# Autodesk Inventor assembly: Cart Assembly
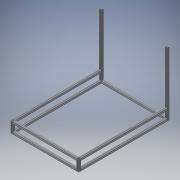
[picture p0: Inventor's stored thumbnail of the model, 180x180]
Saved by Autodesk Inventor 2016 SP2 (Build 200236200, 236)
## iProperties
Created: 2018-02-07
Part Number: Cart Assembly
Document SubType Name: Assembly
Designer: CAD
Author: CAD
## Documents named in this file (5)
- C:\Users\CAD\Documents\GitHub\FIRST-ROBOTICS-2018-5436-CAD\Cart\Cart Assembly.iam
- C:\Users\CAD\Documents\GitHub\FIRST-ROBOTICS-2018-5436-CAD\Cart\Horizontal width piece.ipt
- C:\Users\CAD\Documents\GitHub\FIRST-ROBOTICS-2018-5436-CAD\Cart\Horizontal pice.ipt
- C:\Users\CAD\Documents\GitHub\FIRST-ROBOTICS-2018-5436-CAD\Cart\Vertical piece Handle side.ipt
- C:\Users\CAD\Documents\GitHub\FIRST-ROBOTICS-2018-5436-CAD\Cart\Vertical Piece front side.ipt
## Components (11 placed, 4 different names)
1. Horizontal width piece:1 — Flush:13, Flush:14, Flush:15, Mate:8
2. Horizontal width piece:2 — Mate:2, Flush:3, Flush:4, Flush:5, Flush:6, Mate:3, Flush:8
3. Horizontal pice:1 — Mate:1, Flush:1, Flush:2, Flush:4, Mate:6, Flush:11, Flush:14, Flush:15
4. Horizontal pice:2 — Mate:4, Flush:7, Flush:8, Mate:5, Flush:9, Flush:10
5. Vertical piece Handle side:1 — Mate:5, Flush:9, Flush:10, Flush:12, Mate:7
6. Vertical piece Handle side:2 — Mate:6, Flush:11, Flush:12, Flush:13
7. Vertical Piece front side:1 — Mate:1, Flush:1, Flush:2, Mate:2, Flush:3, Flush:19, Mate:9, Flush:21
8. Vertical Piece front side:2 — Flush:5, Flush:6, Mate:3, Mate:4, Flush:7, Flush:16, Flush:17, Flush:18
9. Horizontal pice:3 — Flush:18, Mate:8, Flush:19, Flush:20
10. Horizontal pice:4 — Flush:16, Mate:7, Flush:17
11. Horizontal width piece:3 — Flush:20, Mate:9, Flush:21
## Relationships (30: Flush 21, Mate 9)
- Mate:1: Horizontal pice:1 ↔ Vertical Piece front side:1
- Flush:1: Horizontal pice:1 ↔ Vertical Piece front side:1
- Flush:2: Horizontal pice:1 ↔ Vertical Piece front side:1
- Mate:2: Horizontal width piece:2 ↔ Vertical Piece front side:1
- Flush:3: Horizontal width piece:2 ↔ Vertical Piece front side:1
- Flush:4: Horizontal width piece:2 ↔ Horizontal pice:1
- Flush:5: Horizontal width piece:2 ↔ Vertical Piece front side:2
- Flush:6: Horizontal width piece:2 ↔ Vertical Piece front side:2
- Mate:3: Horizontal width piece:2 ↔ Vertical Piece front side:2
- Mate:4: Horizontal pice:2 ↔ Vertical Piece front side:2
- Flush:7: Horizontal pice:2 ↔ Vertical Piece front side:2
- Flush:8: Horizontal width piece:2 ↔ Horizontal pice:2
- Mate:5: Horizontal pice:2 ↔ Vertical piece Handle side:1
- Flush:9: Horizontal pice:2 ↔ Vertical piece Handle side:1
- Flush:10: Horizontal pice:2 ↔ Vertical piece Handle side:1
- Mate:6: Horizontal pice:1 ↔ Vertical piece Handle side:2
- Flush:11: Horizontal pice:1 ↔ Vertical piece Handle side:2
- Flush:12: Vertical piece Handle side:1 ↔ Vertical piece Handle side:2
- Flush:13: Horizontal width piece:1 ↔ Vertical piece Handle side:2
- Flush:14: Horizontal width piece:1 ↔ Horizontal pice:1
- Flush:15: Horizontal width piece:1 ↔ Horizontal pice:1
- Flush:16: Vertical Piece front side:2 ↔ Horizontal pice:4
- Mate:7: Vertical piece Handle side:1 ↔ Horizontal pice:4
- Flush:17: Vertical Piece front side:2 ↔ Horizontal pice:4
- Flush:18: Vertical Piece front side:2 ↔ Horizontal pice:3
- Mate:8: Horizontal width piece:1 ↔ Horizontal pice:3
- Flush:19: Vertical Piece front side:1 ↔ Horizontal pice:3
- Flush:20: Horizontal pice:3 ↔ Horizontal width piece:3
- Mate:9: Vertical Piece front side:1 ↔ Horizontal width piece:3
- Flush:21: Vertical Piece front side:1 ↔ Horizontal width piece:3
